# Autodesk Inventor assembly: E002-Piston
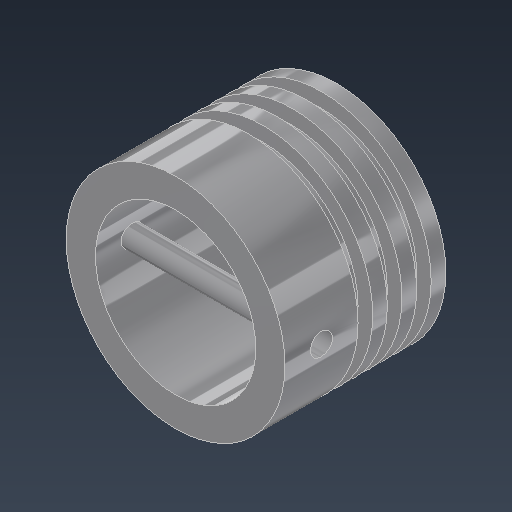
[picture p0: Inventor's stored thumbnail of the model, 512x512]
Saved by Autodesk Inventor 2021.3 (Build 253353000, 353)
## iProperties
Created: 2022-03-31
Part Number: E002-Piston
Document SubType Name: Assembly
Designer: remi
Mass: 22.0129 g
Surface Area: 59.3913 cm^2
Volume: 8.15292 cm^3
Density: 2.7 g/cm^3
Author: remi
## Documents named in this file (3)
- C:\Users\remi\OneDrive\Documents\Cours\05-HEVS\S2fb\mechanic\CCo\project\Compressor\E002-Piston.iam
- C:\Users\remi\OneDrive\Documents\Cours\05-HEVS\S2fb\mechanic\CCo\project\Compressor\P003-Corps_piston.ipt
- C:\Users\remi\OneDrive\Documents\Cours\05-HEVS\S2fb\mechanic\CCo\project\Compressor\P005-Axe_piston.ipt
## Components (2 placed, 2 different names)
1. P003-Corps_piston:1 — Mate:1
2. P005-Axe_piston:1 — Mate:1
## Relationships (1: Mate 1)
- Mate:1: P003-Corps_piston:1 ↔ P005-Axe_piston:1
